# Autodesk Inventor assembly: XCarriageLowTest
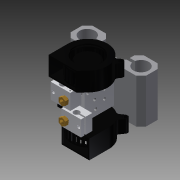
[picture p0: Inventor's stored thumbnail of the model, 180x180]
Saved by Autodesk Inventor 2015 SP1 (Build 190203100, 203)
## iProperties
Created: 2015-03-09
Part Number: XCarriageLowTest
Document SubType Name: Assembly
Designer: Jack
Author: Jack
## Documents named in this file (5)
- C:\Users\Jack\ownCloud\Projects\CrossBot\InventorModel\XAxis\XCarriageLowTest.iam
- C:\Users\Jack\ownCloud\Projects\CrossBot\InventorModel\XAxis\ChimeraXCarriageLowTest.ipt
- C:\Users\Jack\ownCloud\Projects\CrossBot\InventorModel\HotEnds\E3DChimera\E3DChimera.iam
- C:\Users\Jack\ownCloud\Projects\CrossBot\InventorModel\Electronics\Fans\FanRadial50mm.ipt
- C:\Users\Jack\ownCloud\Projects\CrossBot\InventorModel\Electronics\Fans\FanRadial40mm.ipt
## Components (6 placed, 4 different names)
1. ChimeraXCarriageLowTest:1 — Mate:1, Mate:2, Mate:3, Angle:1, Angle:2
2. E3DChimera:1 [sub-assembly] — Mate:1, Mate:2, Mate:3, Mate:4, Mate:5, Mate:6, Mate:7
3. FanRadial50mm:1 — Mate:4
4. FanRadial50mm:2 — Angle:1, Mate:5
5. FanRadial40mm:1 — Mate:6
6. FanRadial40mm:2 — Mate:7, Angle:2
## Relationships (9: Mate 7, Angle 2)
- Mate:1: ChimeraXCarriageLowTest:1 ↔ E3DChimera:1
- Mate:2: ChimeraXCarriageLowTest:1 ↔ E3DChimera:1
- Mate:3: ChimeraXCarriageLowTest:1 ↔ E3DChimera:1
- Angle:1 (0 deg): ChimeraXCarriageLowTest:1 ↔ FanRadial50mm:2
- Mate:4: E3DChimera:1 ↔ FanRadial50mm:1
- Mate:5: E3DChimera:1 ↔ FanRadial50mm:2
- Mate:6: E3DChimera:1 ↔ FanRadial40mm:1
- Mate:7: E3DChimera:1 ↔ FanRadial40mm:2
- Angle:2 (180 deg): ChimeraXCarriageLowTest:1 ↔ FanRadial40mm:2
